# Autodesk Inventor assembly: Drinkmixer
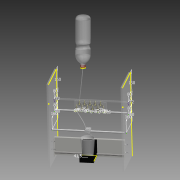
[picture p0: Inventor's stored thumbnail of the model, 180x180]
Saved by Autodesk Inventor 2013 (Build 170138000, 138)
## iProperties
Created: 2012-07-24
Part Number: Drinkmixer
Document SubType Name: Assembly
Designer: fivef
Author: fivef
## Documents named in this file (17)
- D:\Dropbox\My Dropbox\Dokumente\Aktuell\Drinkmixer\Drinkmixer.iam
- D:\Dropbox\My Dropbox\Dokumente\Aktuell\Drinkmixer\Ventilhalter.ipt
- D:\Dropbox\My Dropbox\Dokumente\Aktuell\Drinkmixer\Ventil.ipt
- D:\Dropbox\My Dropbox\Dokumente\Aktuell\Drinkmixer\Schlauchhalter.ipt
- D:\Dropbox\My Dropbox\Dokumente\Aktuell\Drinkmixer\Spanplatten Gehäuse.ipt
- D:\Dropbox\My Dropbox\Dokumente\Aktuell\Drinkmixer\Drinkmixer.Rohr- und Leitungsverläufe01.iam
- D:\Dropbox\My Dropbox\Dokumente\Aktuell\Drinkmixer\Abtropfgitter.ipt
- D:\Dropbox\My Dropbox\Dokumente\Aktuell\Drinkmixer\whiskey glass .ipt
- D:\Dropbox\My Dropbox\Dokumente\Aktuell\Drinkmixer\Flasche.iam
- D:\Dropbox\My Dropbox\Dokumente\Aktuell\Drinkmixer\CocktailGlas.ipt
- D:\Dropbox\My Dropbox\Dokumente\Aktuell\Drinkmixer\Gehäuse.iam
- D:\Dropbox\My Dropbox\Dokumente\Aktuell\Drinkmixer\Glas Drucker Horizontal.iam
- D:\Dropbox\My Dropbox\Dokumente\Aktuell\Drinkmixer\abstandshalter.ipt
- C:\Users\fivef\Documents\Inventor\Content Center Files\R2013\de-DE\DIN 7991(2)\DIN 7991 - M4x25.ipt
- C:\Users\fivef\Documents\Inventor\Content Center Files\R2013\de-DE\DIN 7984\DIN 7984 - M3 x 20.ipt
- C:\Users\fivef\Documents\Inventor\Content Center Files\R2013\de-DE\ISO 4035(1)\ISO 4035 - M3DIN EN.ipt
- C:\Users\fivef\Documents\Inventor\Content Center Files\R2013\de-DE\DIN 914\DIN 914 - M4 x 4.ipt
## Components (44 placed, 16 different names)
1. Ventilhalter:1 — Einfügen:1, Einfügen:2, Einfügen:3, Einfügen:4, Einfügen:5, Einfügen:6, Einfügen:7, Einfügen:8, Einfügen:9, Einfügen:10, Einfügen:11, Passend:60, Passend:61, Passend:63, Passend:70, Passend:71, Passend:74, Passend:75, Passend:76, Passend:77, Passend:78
2. Schlauchhalter:1 — Passend:15, Passend:16, Passend:17, Passend:18, Passend:19
3. Spanplatten Gehäuse:1 — Fluchtend:1, Passend:5, Passend:6
4. Verlauf der Rohre und Leitungen 01 [sub-assembly]
5. Abtropfgitter:1 — Fluchtend:1, Passend:5, Passend:6, Passend:7, Tangential:1, Fluchtend:2
6. whiskey glass :1 — Passend:7, Tangential:1
7. Flasche:2 [sub-assembly]
8. CocktailGlas:1 — Fluchtend:2, Passend:35, Passend:36
9. Gehäuse:1 [sub-assembly] — Passend:15, Passend:16, Passend:17, Passend:29, Passend:33, Passend:34, Passend:37, Passend:38, Passend:39, Passend:40, Passend:41, Passend:42, Passend:43, Einfügen:12, Einfügen:13, Einfügen:14, Einfügen:15, Passend:76, Passend:77, Passend:78
10. DIN 7991 M4x25:1 — Passend:18
11. DIN 7991 M4x25:2 — Passend:19
12. Drucker Horizontal:1 [sub-assembly] — Passend:35, Passend:36, Passend:42, Passend:43, Passend:49, Passend:51, Passend:53, Passend:55
13. abstandshalter:1 — Passend:40, Passend:41
14. abstandshalter:2 — Passend:29, Passend:39
15. abstandshalter:3 — Passend:34, Passend:37
16. abstandshalter:4 — Passend:33, Passend:38
17. Flasche:3 [sub-assembly]
18. Flasche:4 [sub-assembly]
19. DIN 7984 M3 x 20:1 — Einfügen:12, Passend:54
20. DIN 7984 M3 x 20:2 — Einfügen:13, Passend:48
21. DIN 7984 M3 x 20:3 — Einfügen:14, Passend:50
22. DIN 7984 M3 x 20:4 — Einfügen:15, Passend:52
23. DIN EN 24035 M3:3 — Passend:48, Passend:49
24. DIN EN 24035 M3:4 — Passend:50, Passend:51
25. DIN EN 24035 M3:5 — Passend:52, Passend:53
26. DIN EN 24035 M3:6 — Passend:54, Passend:55
27. DIN 914 M4 x 4:7 — Passend:60
28. DIN 914 M4 x 4:8 — Passend:61
29. DIN 914 M4 x 4:9 — Passend:63
30. DIN 914 M4 x 4:1 — Passend:70
31. DIN 914 M4 x 4:2 — Passend:71
32. DIN 914 M4 x 4:5 — Passend:74
33. DIN 914 M4 x 4:6 — Passend:75
34. Ventil:1 — Einfügen:1
35. Ventil:2 — Einfügen:2
36. Ventil:3 — Einfügen:3
37. Ventil:4 — Einfügen:4
38. Ventil:5 — Einfügen:5
39. Ventil:6 — Einfügen:7
40. Ventil:7 — Einfügen:6
41. Ventil:8 — Einfügen:8
42. Ventil:9 — Einfügen:11
43. Ventil:10 — Einfügen:10
44. Ventil:11 — Einfügen:9
## Relationships (59: Mate 38, Insert 15, Flush 5, Tangent 1)
- Einfügen:1 [Insert]: Ventilhalter:1 ↔ Ventil:1
- Einfügen:2 [Insert]: Ventilhalter:1 ↔ Ventil:2
- Einfügen:3 [Insert]: Ventilhalter:1 ↔ Ventil:3
- Einfügen:4 [Insert]: Ventilhalter:1 ↔ Ventil:4
- Einfügen:5 [Insert]: Ventilhalter:1 ↔ Ventil:5
- Einfügen:6 [Insert]: Ventilhalter:1 ↔ Ventil:7
- Einfügen:7 [Insert]: Ventilhalter:1 ↔ Ventil:6
- Einfügen:8 [Insert]: Ventilhalter:1 ↔ Ventil:8
- Einfügen:9 [Insert]: Ventilhalter:1 ↔ Ventil:11
- Einfügen:10 [Insert]: Ventilhalter:1 ↔ Ventil:10
- Einfügen:11 [Insert]: Ventilhalter:1 ↔ Ventil:9
- Fluchtend:1 [Flush]: Spanplatten Gehäuse:1 ↔ Abtropfgitter:1
- Passend:5 [Mate] (-10 mm): Spanplatten Gehäuse:1 ↔ Abtropfgitter:1
- Passend:6 [Mate] (-10 mm): Spanplatten Gehäuse:1 ↔ Abtropfgitter:1
- Passend:7 [Mate]: Abtropfgitter:1 ↔ whiskey glass :1
- Tangential:1: Abtropfgitter:1 ↔ whiskey glass :1
- Fluchtend:2 [Flush]: Abtropfgitter:1 ↔ CocktailGlas:1
- Passend:15 [Mate]: Schlauchhalter:1 ↔ Gehäuse:1
- Passend:16 [Mate]: Schlauchhalter:1 ↔ Gehäuse:1
- Passend:17 [Mate]: Schlauchhalter:1 ↔ Gehäuse:1
- [Flush]: Drucker Horizontal:1
- Fluchtend:7 [Flush]
- Passend:29 [Mate]: Gehäuse:1 ↔ abstandshalter:2
- Passend:33 [Mate]: Gehäuse:1 ↔ abstandshalter:4
- Passend:34 [Mate]: Gehäuse:1 ↔ abstandshalter:3
- [Flush]: Drucker Horizontal:1
- Passend:35 [Mate]: CocktailGlas:1 ↔ Drucker Horizontal:1
- Passend:36 [Mate]: CocktailGlas:1 ↔ Drucker Horizontal:1
- Passend:37 [Mate]: Gehäuse:1 ↔ abstandshalter:3
- Passend:38 [Mate]: Gehäuse:1 ↔ abstandshalter:4
- Passend:39 [Mate]: Gehäuse:1 ↔ abstandshalter:2
- Passend:40 [Mate]: Gehäuse:1 ↔ abstandshalter:1
- Passend:41 [Mate]: Gehäuse:1 ↔ abstandshalter:1
- Passend:42 [Mate]: Gehäuse:1 ↔ Drucker Horizontal:1
- Passend:43 [Mate]: Gehäuse:1 ↔ Drucker Horizontal:1
- Passend:49 [Mate]: Drucker Horizontal:1 ↔ DIN EN 24035 M3:3
- Passend:51 [Mate]: Drucker Horizontal:1 ↔ DIN EN 24035 M3:4
- Passend:53 [Mate]: Drucker Horizontal:1 ↔ DIN EN 24035 M3:5
- Passend:55 [Mate]: Drucker Horizontal:1 ↔ DIN EN 24035 M3:6
- Passend:76 [Mate]: Ventilhalter:1 ↔ Gehäuse:1
- Passend:77 [Mate]: Ventilhalter:1 ↔ Gehäuse:1
- Passend:78 [Mate]: Ventilhalter:1 ↔ Gehäuse:1
- Passend:18 [Mate]: Schlauchhalter:1 ↔ DIN 7991 M4x25:1
- Passend:19 [Mate]: Schlauchhalter:1 ↔ DIN 7991 M4x25:2
- Einfügen:12 [Insert]: Gehäuse:1 ↔ DIN 7984 M3 x 20:1
- Einfügen:13 [Insert]: Gehäuse:1 ↔ DIN 7984 M3 x 20:2
- Einfügen:14 [Insert]: Gehäuse:1 ↔ DIN 7984 M3 x 20:3
- Einfügen:15 [Insert]: Gehäuse:1 ↔ DIN 7984 M3 x 20:4
- Passend:48 [Mate]: DIN 7984 M3 x 20:2 ↔ DIN EN 24035 M3:3
- Passend:50 [Mate]: DIN 7984 M3 x 20:3 ↔ DIN EN 24035 M3:4
- Passend:52 [Mate]: DIN 7984 M3 x 20:4 ↔ DIN EN 24035 M3:5
- Passend:54 [Mate]: DIN 7984 M3 x 20:1 ↔ DIN EN 24035 M3:6
- Passend:60 [Mate]: Ventilhalter:1 ↔ DIN 914 M4 x 4:7
- Passend:61 [Mate]: Ventilhalter:1 ↔ DIN 914 M4 x 4:8
- Passend:63 [Mate]: Ventilhalter:1 ↔ DIN 914 M4 x 4:9
- Passend:70 [Mate]: Ventilhalter:1 ↔ DIN 914 M4 x 4:1
- Passend:71 [Mate]: Ventilhalter:1 ↔ DIN 914 M4 x 4:2
- Passend:74 [Mate]: Ventilhalter:1 ↔ DIN 914 M4 x 4:5
- Passend:75 [Mate]: Ventilhalter:1 ↔ DIN 914 M4 x 4:6
